# Autodesk Inventor assembly: .375'' Screw & Nylock Nut
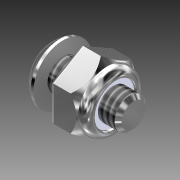
[picture p0: Inventor's stored thumbnail of the model, 180x180]
Saved by Autodesk Inventor 2012 (Build 160160000, 160)
## iProperties
Created: 2011-09-11
Part Number: .375'' Screw & Nylock Nut
Document SubType Name: Assembly
Designer: Wade
Author: Wade
## Documents named in this file (3)
- C:\Users\Wade\Documents\1103 Robot - CAD Assembly\.375'' Screw & Nylock Nut.iam
- C:\Users\Wade\Documents\24C VEX CAD Files\Screws & Nuts\Screw 8-32 x 0.375''-Silver.ipt
- C:\Users\Wade\Documents\24C VEX CAD Files\Screws & Nuts\Nut 8-32 Nylock.ipt
## Components (2 placed, 2 different names)
1. Screw 8-32 x 0.375''-Silver:1 — Mate:1, Mate:2
2. Nut 8-32 Nylock:1 — Mate:1, Mate:2
## Relationships (2: Mate 2)
- Mate:1: Screw 8-32 x 0.375''-Silver:1 ↔ Nut 8-32 Nylock:1
- Mate:2 (2.3368 mm): Screw 8-32 x 0.375''-Silver:1 ↔ Nut 8-32 Nylock:1
